# Autodesk Inventor assembly: HBLFSNK5-C-SEP
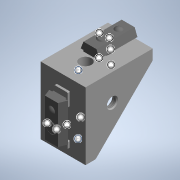
[picture p0: Inventor's stored thumbnail of the model, 180x180]
Saved by Autodesk Inventor 2022 (Build 260153000, 153)
## iProperties
Category: PARTsolutions
Company: MISUMI
Part Number: HBLFSNK5-C-SEP
Catalog Web Link: www.cadenas.de
Description: HBLFSN5, HBLFSN5-4, HBLFSNB5, HBLFSNM5, HBLFSNK5, HBLFSNE5-Brackets HFS5 Reversal Brackets with Tab
Vendor: MISUMI
Document SubType Name: Assembly
Designer: partserver
Manufacturer: MISUMI
Mass: 7.78214 g
Surface Area: 60.4641 cm^2
Volume: 7.78214 cm^3
Density: 1 g/cm^3
PSOL_IDENT_0: {$CADENAS_DATA\23d-libs\misumi\metric\38_al_extrusions_blackets\5\hblfsnm5_asmtab.prj},234 {VTYP=3D}
PSOL_IDENT_1: ,{STYP=ASSTAB},{NB=HBLFSNK5-C-SEP},{LINA=HBLFSNK5-C-SEP},{NN=HBLFSN5, HBLFSN5-4, HBLFSNB5, HBLFSNM5,
PSOL_IDENT_2: HBLFSNK5, HBLFSNE5},{DATE=30.06.2021 13:16:08},{GEOMDATE=14.12.2010},{VERSION=},{LINEID=40},{WBVAR=
PSOL_IDENT_3: ALT1,ALT2},{WBNUMERIC=}  {NB=HBLFSNK5-C-SEP},{LINA=HBLFSNK5-C-SEP},{KT=5},{PN=HBLFSNK5-C-SEP},{TP=HB
PSOL_IDENT_4: LFSNK5},{NOH=1},{NOHV=2},{MAT=ADC12},{ST=-},{TYPE=HBLFSNK5},{FEAT=Bracket with Single Side Tab},{ALT
PSOL_IDENT_5: 1=-C},{ALT2=-SEP},{MASS=15},{AB=CBM5-10},{NOB=2},{AN=HNTP5-5},{NON=2},{AL=1176},{W=20},{H=30},{DP=30
PSOL_IDENT_6: },{T=5.0},{HDIS=8},{DPOS=12},{HH1=18},{HV1=10},{DIA=5.2},{ALT1ALG='','w/o C (Mounting Holes for Cove
PSOL_IDENT_7: r)','-C','with C (Mounting Holes for Cover)'},{ALT2ALG= '' , 'w/o Set Applicable Bolt & Nut' , '-SET'
PSOL_IDENT_8: , 'with SET (Set Applicable Bolt & Nut)' , '-SST' , 'with SST (Stainless Steel Set Applicable Bolt
PSOL_IDENT_9: & Nut)' , '-SEU' , 'with SEU (Pre-Assy. Insertion Spring Nuts Set Applicable Bolt & Nut)' , '-SSU' ,
PSOL_IDENT_10: 'with SSU (Pre-Assy. Insertion Spring Nuts Stainless Steel Set Applicable Bolt & Nut)' , '-SEP' , '
PSOL_IDENT_11: with SEP (Post-Assy. Insertion Spring Nuts Set Applicable Bolt & Nut)' , '-SSP' , 'with SSP (Post-As
PSOL_IDENT_12: sy. Insertion Spring Nuts Set Applicable Bolt & Nut)' },{R=1},{R1=0.3},{APOSV=0},{VER=1},{PR=5},{TT=
PSOL_IDENT_13: 1.0},{T1=2},{TIP=HBLFSN5},{PPATH=hblfsl5_asmtpl.prj},{ABT=CBM5-},{ABL=10}
NB: HBLFSNK5-C-SEP
NN: HBLFSN5, HBLFSN5-4, HBLFSNB5, HBLFSNM5, HBLFSNK5, HBLFSNE5
NT: Brackets HFS5 Reversal Brackets with Tab
NBSYN: $PN.
LINA: HBLFSNK5-C-SEP
CATALOG: Misumi
PN: HBLFSNK5-C-SEP
TP: HBLFSNK5
MAT: ADC12
ST: -
FEAT: Bracket with Single Side Tab
ALT1: with C (Mounting Holes for Cover)
ALT2: with SEP (Post-Assy. Insertion Spring Nuts Set Applicable Bolt & Nut)
MASS: 15
AB: CBM5-10
NOB: 2
AN: HNTP5-5
NON: 2
AL: 1176
SUPPLIER: MISUMI
ARTICLENO: HBLFSNK5-C-SEP
BOMINFO: HBLFSNK5-C-SEP
CREATOR: CADENAS GmbH
Title: HBLFSNK5-C-SEP
Author: Cadenas PARTsolutions
Comments: Brackets HFS5 Reversal Brackets with Tab
## Documents named in this file (4)
- C:\Users\yuto6\Box\Public_Share\キャチロボバトルコンテスト2021\CAD\catchrobo_hardware\assy-shooter\HBLFSNK5-C-SEP.iam
- C:\Users\yuto6\Box\Public_Share\キャチロボバトルコンテスト2021\CAD\catchrobo_hardware\assy-shooter\HBLFSNK5-C-SEPh5.ipt
- C:\Users\yuto6\Box\Public_Share\キャチロボバトルコンテスト2021\CAD\catchrobo_hardware\assy-shooter\CBM5-10.ipt
- C:\Users\yuto6\Box\Public_Share\キャチロボバトルコンテスト2021\CAD\catchrobo_hardware\assy-shooter\HNTP5-5_app.ipt
## Components (5 placed, 3 different names)
1. HBLFSNK5-C-SEPh5:1 — to_bolt_row_4_to_7_Z@1 <-> bolt_Z@2, to_nut_row_4_to_7_Z@1 <-> to_frames_Z@3, to_bolt_4_7_base_Z@1 <-> bolt_Z@4, to_nut_base_4_7_Z@1 <-> to_frames_Z@5
2. CBM5-10:1 — to_bolt_row_4_to_7_Z@1 <-> bolt_Z@2
3. HNTP5-5_app:1 — to_nut_row_4_to_7_Z@1 <-> to_frames_Z@3
4. CBM5-10:2 — to_bolt_4_7_base_Z@1 <-> bolt_Z@4
5. HNTP5-5_app:2 — to_nut_base_4_7_Z@1 <-> to_frames_Z@5
## Relationships (4: Mate 4)
- to_bolt_row_4_to_7_Z@1 <-> bolt_Z@2 [Mate]: HBLFSNK5-C-SEPh5:1 ↔ CBM5-10:1
- to_nut_row_4_to_7_Z@1 <-> to_frames_Z@3 [Mate]: HBLFSNK5-C-SEPh5:1 ↔ HNTP5-5_app:1
- to_bolt_4_7_base_Z@1 <-> bolt_Z@4 [Mate]: HBLFSNK5-C-SEPh5:1 ↔ CBM5-10:2
- to_nut_base_4_7_Z@1 <-> to_frames_Z@5 [Mate]: HBLFSNK5-C-SEPh5:1 ↔ HNTP5-5_app:2
